# Autodesk Inventor assembly: Assembly
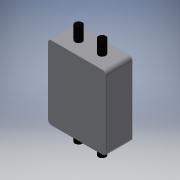
[picture p0: Inventor's stored thumbnail of the model, 180x180]
Saved by Autodesk Inventor 2016 (Build 200138000, 138)
## iProperties
Created: 2016-03-25
Part Number: Assembly
Document SubType Name: Assembly
Designer: Paschalis
Author: Paschalis
## Documents named in this file (4)
- C:\Users\Paschalis\Documents\eagle\Measuring-PCB\3D\Assembly.iam
- C:\Users\Paschalis\Documents\eagle\Measuring-PCB\3D\box_base.ipt
- C:\Users\Paschalis\Documents\eagle\Measuring-PCB\3D\board2.brd.iam
- C:\Users\Paschalis\Documents\eagle\Measuring-PCB\3D\MC4_plug.ipt
## Components (6 placed, 3 different names)
1. box_base:1 — Mate:1, Mate:2, Mate:3, Mate:4, Mate:5, Mate:6, Mate:7, Mate:8, Mate:9, Mate:10, Mate:11
2. board2.brd:1 [sub-assembly] — Mate:1, Mate:2, Mate:3
3. MC4_plug:1 — Mate:4, Mate:8
4. MC4_plug:2 — Mate:6, Mate:10
5. MC4_plug:3 — Mate:5, Mate:9
6. MC4_plug:4 — Mate:7, Mate:11
## Relationships (11: Mate 11)
- Mate:1 (5 mm): box_base:1 ↔ board2.brd:1
- Mate:2 (20 mm): box_base:1 ↔ board2.brd:1
- Mate:3 (10 mm): box_base:1 ↔ board2.brd:1
- Mate:4: box_base:1 ↔ MC4_plug:1
- Mate:5: box_base:1 ↔ MC4_plug:3
- Mate:6: box_base:1 ↔ MC4_plug:2
- Mate:7: box_base:1 ↔ MC4_plug:4
- Mate:8: box_base:1 ↔ MC4_plug:1
- Mate:9: box_base:1 ↔ MC4_plug:3
- Mate:10: box_base:1 ↔ MC4_plug:2
- Mate:11: box_base:1 ↔ MC4_plug:4
